# Autodesk Inventor assembly: LED Bar
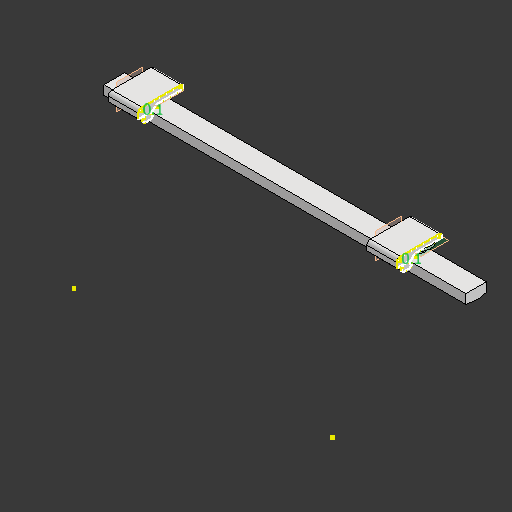
[picture p0: Inventor's stored thumbnail of the model, 512x512]
Saved by Autodesk Inventor 2023 (Build 270158000, 158)
## iProperties
Created: 2023-01-05
Part Number: LED Bar
Document SubType Name: Assembly
Designer: alber
Author: alber
## Documents named in this file (4)
- C:\Users\alber\Desktop\Files\Ender3-Upgrade\CAD\LED Bar.iam
- C:\Users\alber\Desktop\Files\Ender3-Upgrade\CAD\Led Light.ipt
- C:\Users\alber\Desktop\Files\Ender3-Upgrade\CAD\LED Holder.ipt
- C:\Users\alber\Desktop\Files\Ender3-Upgrade\CAD\LED Holder Magnetic.ipt
## Components (5 placed, 3 different names)
1. Led Light:1
2. LED Holder:1
3. LED Holder Magnetic:1
4. LED Holder Magnetic:2
5. LED Holder:2
## Relationships (5: Flush 4, Mate 1)
- [Flush]: LED Holder:1 ↔ LED Holder Magnetic:1
- [Flush]: LED Holder:1 ↔ LED Holder Magnetic:1
- [Flush]: LED Holder Magnetic:2 ↔ LED Holder:2
- [Flush]: LED Holder:1 ↔ LED Holder:2
- [Mate]: LED Holder Magnetic:2 ↔ LED Holder:2
## Named parameters: d2_d4 = 0 mm
